# Autodesk Inventor assembly: KrakenCustom
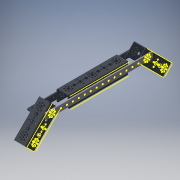
[picture p0: Inventor's stored thumbnail of the model, 180x180]
Saved by Autodesk Inventor 2016 (Build 200138000, 138)
## iProperties
Created: 2015-09-12
Part Number: KrakenCustom
Document SubType Name: Assembly
Designer: Tim
Author: Tim
## Documents named in this file (5)
- C:\Users\Tim\Documents\GitHub\phi_robotics\3d-models\FTC_Tetrix_KOP_Block_Party\Tim Bloot Designs\KrakenCustom.iam
- C:\Users\Tim\Documents\GitHub\phi_robotics\3d-models\FTC_Tetrix_KOP_Block_Party\Tetrix_Kit_FTC\Autodesk Inventor Files\tetrix_angle-288 MM.ipt
- C:\Users\Tim\Documents\GitHub\phi_robotics\3d-models\FTC_Tetrix_KOP_Block_Party\Tetrix_Kit_FTC\Autodesk Inventor Files\tetrix_flat_bar-288 MM.ipt
- C:\Users\Tim\Documents\GitHub\phi_robotics\3d-models\FTC_Tetrix_KOP_Block_Party\Tetrix_Kit_FTC\Autodesk Inventor Files\tetrix_c_channel-2.ipt
- C:\Users\Tim\Documents\GitHub\phi_robotics\3d-models\FTC_Tetrix_KOP_Block_Party\Tetrix_Kit_FTC\Autodesk Inventor Files\tetrix_c_channel-3.ipt
## Components (5 placed, 4 different names)
1. tetrix_angle-288 MM:1
2. tetrix_flat_bar-288 MM:1
3. tetrix_c_channel-2:1
4. tetrix_c_channel-2:2
5. tetrix_c_channel-3:1
## Relationships (5: WeldJoint 5)
- [WeldJoint]: tetrix_flat_bar-288 MM:1 ↔ tetrix_c_channel-2:1
- [WeldJoint]: tetrix_flat_bar-288 MM:1 ↔ tetrix_c_channel-2:2
- [WeldJoint]: tetrix_angle-288 MM:1 ↔ tetrix_c_channel-2:2
- [WeldJoint]: tetrix_angle-288 MM:1 ↔ tetrix_c_channel-2:1
- [WeldJoint]: tetrix_flat_bar-288 MM:1 ↔ tetrix_c_channel-3:1
## Named parameters: d0_d2 = 0 mm, d1_d3 = 0 mm
